# Autodesk Inventor assembly: wedge
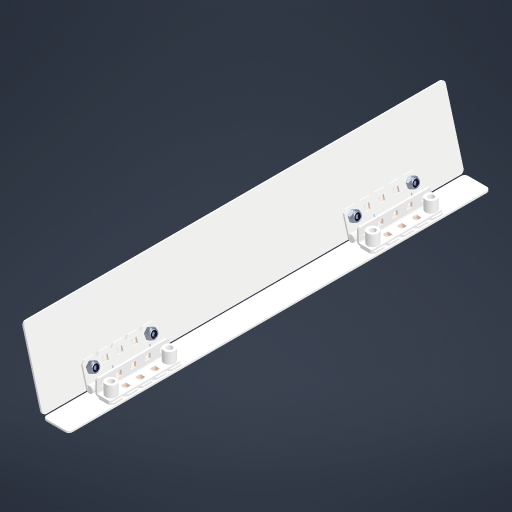
[picture p0: Inventor's stored thumbnail of the model, 512x512]
Saved by Autodesk Inventor 2023 (Build 270158000, 158)
## iProperties
Created: 2023-08-07
Part Number: wedge
Document SubType Name: Assembly
Designer: srbel
Author: srbel
## Documents named in this file (10)
- C:\CAD\OverUnderCAD\Drive\wedge.iam
- C:\CAD Robotics Season 23-24\top of wedge.ipt
- C:\CAD\OverUnderCAD\VEX-CAD-Inventor-1.4.0\Structure\Angle\Aluminum\1x1\Alu Angle 1x1x5.ipt
- C:\CAD\OverUnderCAD\VEX-CAD-Inventor-1.4.0\Motion\Spacers\Spacer Nylon .313 OD\NSpacer .313 OD x .375.ipt
- C:\CAD\OverUnderCAD\VEX-CAD-Inventor-1.4.0\Motion\Spacers\Spacer Nylon .313 OD.ipt
- C:\CAD\OverUnderCAD\VEX-CAD-Inventor-1.4.0\Motion\Hinges\Hinge 5 Holes.iam
- C:\CAD Robotics Season 23-24\wedge.ipt
- C:\CAD\OverUnderCAD\VEX-CAD-Inventor-1.4.0\Structure\Hardware\Screw Steel - Star\SScrew Star Threaded .250.ipt
- C:\CAD\OverUnderCAD\VEX-CAD-Inventor-1.4.0\Structure\Hardware\Screw Steel - Star.ipt
- C:\CAD\OverUnderCAD\VEX-CAD-Inventor-1.4.0\Structure\Hardware\Nut Thin Nylock.ipt
## Components (18 placed, 7 different names)
1. Alu Angle 1x1x5:1 — Insert:9, Insert:10, Insert:13, Insert:14
2. Alu Angle 1x1x5:2 — Insert:11, Insert:12, Insert:15, Insert:16
3. NSpacer .313 OD x .375:1 — Insert:9
4. NSpacer .313 OD x .375:2 — Insert:10
5. NSpacer .313 OD x .375:3 — Insert:11
6. NSpacer .313 OD x .375:4 — Insert:12
7. Hinge 5 Holes:1 [sub-assembly] — Insert:13, Insert:14, Insert:19, Insert:22, Insert:27, Insert:28
8. Hinge 5 Holes:2 [sub-assembly] — Insert:15, Insert:16, Insert:20, Insert:21, Insert:29, Insert:30
9. wedge:1 — Insert:19, Insert:20, Insert:23, Insert:24, Insert:25, Insert:26
10. top of wedge:1 — Insert:21, Insert:22
11. SScrew Star Threaded .250:1 — Insert:23
12. SScrew Star Threaded .250:2 — Insert:24
13. SScrew Star Threaded .250:3 — Insert:25
14. SScrew Star Threaded .250:4 — Insert:26
15. Nut Thin Nylock:1 — Insert:28
16. Nut Thin Nylock:2 — Insert:29
17. Nut Thin Nylock:3 — Insert:30
18. Nut Thin Nylock:4 — Insert:27
## Relationships (20: Insert 20)
- Insert:9: Alu Angle 1x1x5:1 ↔ NSpacer .313 OD x .375:1
- Insert:10: Alu Angle 1x1x5:1 ↔ NSpacer .313 OD x .375:2
- Insert:11: Alu Angle 1x1x5:2 ↔ NSpacer .313 OD x .375:3
- Insert:12: Alu Angle 1x1x5:2 ↔ NSpacer .313 OD x .375:4
- Insert:13: Alu Angle 1x1x5:1 ↔ Hinge 5 Holes:1
- Insert:14: Alu Angle 1x1x5:1 ↔ Hinge 5 Holes:1
- Insert:15: Alu Angle 1x1x5:2 ↔ Hinge 5 Holes:2
- Insert:16: Alu Angle 1x1x5:2 ↔ Hinge 5 Holes:2
- Insert:19: Hinge 5 Holes:1 ↔ wedge:1
- Insert:20: Hinge 5 Holes:2 ↔ wedge:1
- Insert:21: Hinge 5 Holes:2 ↔ top of wedge:1
- Insert:22: Hinge 5 Holes:1 ↔ top of wedge:1
- Insert:23: wedge:1 ↔ SScrew Star Threaded .250:1
- Insert:24: wedge:1 ↔ SScrew Star Threaded .250:2
- Insert:25: wedge:1 ↔ SScrew Star Threaded .250:3
- Insert:26: wedge:1 ↔ SScrew Star Threaded .250:4
- Insert:27: Hinge 5 Holes:1 ↔ Nut Thin Nylock:4
- Insert:28: Hinge 5 Holes:1 ↔ Nut Thin Nylock:1
- Insert:29: Hinge 5 Holes:2 ↔ Nut Thin Nylock:2
- Insert:30: Hinge 5 Holes:2 ↔ Nut Thin Nylock:3
